# Autodesk Inventor assembly: Tarot 810 Reverse
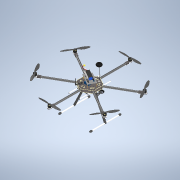
[picture p0: Inventor's stored thumbnail of the model, 180x180]
Saved by Autodesk Inventor 2020 (Build 240168000, 168)
## iProperties
Created: 2020-04-17
Part Number: Tarot 810 Reverse
Document SubType Name: Assembly
Designer: Muhyidin
Author: Muhyidin
## Documents named in this file (20)
- D:\ITS\BAYUCARAKA\PROYEK '19 - '20\Tarot 810\Tarot 810 Reverse.iam
- D:\ITS\BAYUCARAKA\PROYEK '19 - '20\Tarot 810\FRAME ATAS.ipt
- D:\ITS\BAYUCARAKA\PROYEK '19 - '20\Tarot 810\Arem2.iam
- D:\ITS\BAYUCARAKA\PROYEK '19 - '20\Tarot 810\FRAME BAWAH.ipt
- D:\ITS\BAYUCARAKA\PROYEK '19 - '20\Tarot 810\retractable-landing-gear-octocopter-1.snapshot.9\retract assy.iam
- D:\ITS\BAYUCARAKA\PROYEK '19 - '20\Tarot 810\ganjalan landing gear.ipt
- D:\ITS\BAYUCARAKA\PROYEK '19 - '20\Tarot 810\T-Motor U5.ipt
- D:\ITS\BAYUCARAKA\PROYEK '19 - '20\Tarot 810\antena_arm.ipt
- D:\ITS\BAYUCARAKA\PROYEK '19 - '20\Tarot 810\antena_GPS.ipt
- D:\ITS\BAYUCARAKA\PROYEK '19 - '20\Tarot 810\mounting_gps.ipt
- D:\ITS\BAYUCARAKA\PROYEK '19 - '20\Tarot 810\propeler.ipt
- D:\ITS\BAYUCARAKA\PROYEK '19 - '20\Tarot 810\Pixhawk.iam
- D:\ITS\BAYUCARAKA\PROYEK '19 - '20\Tarot 810\Rasberry_box_assembly.iam
- D:\ITS\BAYUCARAKA\PROYEK '19 - '20\Tarot 810\Distans Erkek M3x50mm YP-550.ipt
- D:\ITS\BAYUCARAKA\PROYEK '19 - '20\Tarot 810\Tempat Batere.ipt
- D:\ITS\BAYUCARAKA\PROYEK '19 - '20\Tarot 810\m3.ipt
- D:\ITS\BAYUCARAKA\PROYEK '19 - '20\Tarot 810\Telemetry.iam
- D:\ITS\BAYUCARAKA\PROYEK '19 - '20\Tarot 810\BATERIA.ipt
- D:\ITS\BAYUCARAKA\PROYEK '19 - '20\Tarot 810\bolt_atas.ipt
- D:\ITS\BAYUCARAKA\PROYEK '19 - '20\Tarot 810\mur M3.ipt
## Components (87 placed, 19 different names)
1. FRAME ATAS:1 — Rotational:1, Rotational:2, Rotational:3, Rotational:4, Rotational:5, Rotational:6, Rotational:17, Rotational:26, Rotational:28, Rotational:29, Rotational:30, Rotational:31, Rotational:32, Rigid:1, Rigid:2, Rigid:3, Rigid:4, Rigid:5, Rigid:6, Rigid:7, Rigid:8, Rigid:9, Rigid:10, Rigid:11, Rigid:12, Rigid:13, Rigid:14, Rigid:15, Rigid:16, Rigid:17, Rigid:18, Rigid:19, Rigid:20, Rigid:21, Rigid:22, Rigid:23, Rigid:24, Rigid:25
2. Arem2:1 [sub-assembly] — Rotational:1, Rotational:7, Rotational:12
3. Arem2:2 [sub-assembly] — Rotational:2, Rotational:11
4. Arem2:3 [sub-assembly] — Rotational:3, Rotational:13
5. Arem2:4 [sub-assembly] — Rotational:4, Rotational:14
6. Arem2:5 [sub-assembly] — Rotational:5, Rotational:15
7. Arem2:6 [sub-assembly] — Rotational:6, Rotational:16
8. FRAME BAWAH:1 — Rotational:7, Rotational:8, Rotational:9, Rotational:39, Rotational:40, Rotational:41, Rotational:42, Rotational:43, Rotational:44, Rotational:45, Rotational:46, Rotational:47, Rotational:48, Rotational:49, Rotational:50, Rotational:51, Rotational:52, Rotational:53, Rotational:54, Rotational:55, Rotational:56, Rotational:57, Rotational:58, Rotational:59, Rotational:60, Rotational:61, Rotational:62
9. retract assy:1 [sub-assembly] — Rotational:10
10. ganjalan landing gear:1 — Rotational:8, Rotational:10
11. ganjalan landing gear:2 — Rotational:9
12. T-Motor U5:1 — Rotational:11, Rotational:24
13. T-Motor U5:2 — Rotational:13, Rotational:20
14. T-Motor U5:3 — Rotational:14, Rotational:21
15. T-Motor U5:4 — Rotational:15, Rotational:22
16. T-Motor U5:5 — Rotational:16, Rotational:23
17. T-Motor U5:6 — Rotational:12, Rotational:25
18. antena_arm:1 — Rotational:18, Rotational:19
19. antena_GPS:1 — Rotational:19
20. mounting_gps:1 — Rotational:17, Rotational:18
21. propeler:1 — Rotational:20
22. propeler:2 — Rotational:21
23. propeler:3 — Rotational:22
24. propeler:4 — Rotational:23
25. propeler:5 — Rotational:24
26. propeler:6 — Rotational:25
27. Pixhawk:1 [sub-assembly] — Rotational:27
28. Rasberry_box_assembly:1 [sub-assembly] — Rotational:26, Rotational:27
29. Distans Erkek M3x50mm YP-550:1 — Rotational:28
30. Distans Erkek M3x50mm YP-550:2 — Rotational:29
31. Distans Erkek M3x50mm YP-550:3 — Rotational:31
32. Distans Erkek M3x50mm YP-550:4 — Rotational:30
33. Tempat Batere:1 — Rotational:32, Rotational:33, Rotational:34, Rotational:35, Rotational:36, Rotational:63
34. m3:1 — Rotational:35
35. m3:2 — Rotational:36
36. m3:3 — Rotational:34
37. m3:4 — Rotational:33
38. bolt_atas:1 — Rigid:12
39. bolt_atas:2 — Rigid:11
40. bolt_atas:3 — Rigid:9
41. bolt_atas:4 — Rigid:10
42. bolt_atas:5 — Rigid:8
43. bolt_atas:6 — Rigid:7
44. bolt_atas:7 — Rigid:6
45. bolt_atas:8 — Rigid:4
46. bolt_atas:9 — Rigid:5
47. bolt_atas:10 — Rigid:1
48. bolt_atas:11 — Rigid:3
49. bolt_atas:12 — Rigid:2
50. bolt_atas:13 — Rigid:13
51. bolt_atas:14 — Rigid:14
52. bolt_atas:15 — Rigid:15
53. bolt_atas:16 — Rigid:16
54. bolt_atas:17 — Rigid:17
55. bolt_atas:18 — Rigid:18
56. bolt_atas:19 — Rigid:19
57. bolt_atas:20 — Rigid:20
58. bolt_atas:21 — Rigid:21
59. bolt_atas:22 — Rigid:22
60. bolt_atas:23 — Rigid:23
61. bolt_atas:24 — Rigid:24
62. Telemetry:1 [sub-assembly] — Rigid:25
63. mur M3:1 — Rotational:41
64. mur M3:2 — Rotational:45
65. mur M3:3 — Rotational:50
66. mur M3:4 — Rotational:51
67. mur M3:5 — Rotational:46
68. mur M3:6 — Rotational:44
69. mur M3:7 — Rotational:57
70. mur M3:8 — Rotational:62
71. mur M3:9 — Rotational:59
72. mur M3:10 — Rotational:61
73. mur M3:11 — Rotational:47
74. mur M3:12 — Rotational:39
75. mur M3:13 — Rotational:40
76. mur M3:14 — Rotational:49
77. mur M3:16 — Rotational:58
78. mur M3:17 — Rotational:56
79. mur M3:18 — Rotational:53
80. mur M3:19 — Rotational:55
81. mur M3:21 — Rotational:60
82. mur M3:22 — Rotational:42
83. mur M3:23 — Rotational:43
84. mur M3:24 — Rotational:48
85. mur M3:25 — Rotational:54
86. mur M3:26 — Rotational:52
87. BATERIA:1 — Rotational:63
## Relationships (86: RevoluteJoint 61, WeldJoint 25)
- Rotational:1 [RevoluteJoint]: FRAME ATAS:1 ↔ Arem2:1
- Rotational:2 [RevoluteJoint]: FRAME ATAS:1 ↔ Arem2:2
- Rotational:3 [RevoluteJoint]: FRAME ATAS:1 ↔ Arem2:3
- Rotational:4 [RevoluteJoint]: FRAME ATAS:1 ↔ Arem2:4
- Rotational:5 [RevoluteJoint]: FRAME ATAS:1 ↔ Arem2:5
- Rotational:6 [RevoluteJoint]: FRAME ATAS:1 ↔ Arem2:6
- Rotational:7 [RevoluteJoint]: Arem2:1 ↔ FRAME BAWAH:1
- Rotational:8 [RevoluteJoint]: FRAME BAWAH:1 ↔ ganjalan landing gear:1
- Rotational:9 [RevoluteJoint]: FRAME BAWAH:1 ↔ ganjalan landing gear:2
- Rotational:10 [RevoluteJoint]: retract assy:1 ↔ ganjalan landing gear:1
- Rotational:11 [RevoluteJoint]: Arem2:2 ↔ T-Motor U5:1
- Rotational:12 [RevoluteJoint]: Arem2:1 ↔ T-Motor U5:6
- Rotational:13 [RevoluteJoint]: Arem2:3 ↔ T-Motor U5:2
- Rotational:14 [RevoluteJoint]: Arem2:4 ↔ T-Motor U5:3
- Rotational:15 [RevoluteJoint]: Arem2:5 ↔ T-Motor U5:4
- Rotational:16 [RevoluteJoint]: Arem2:6 ↔ T-Motor U5:5
- Rotational:17 [RevoluteJoint]: FRAME ATAS:1 ↔ mounting_gps:1
- Rotational:18 [RevoluteJoint]: antena_arm:1 ↔ mounting_gps:1
- Rotational:19 [RevoluteJoint] (-15 mm): antena_arm:1 ↔ antena_GPS:1
- Rotational:20 [RevoluteJoint]: T-Motor U5:2 ↔ propeler:1
- Rotational:21 [RevoluteJoint]: T-Motor U5:3 ↔ propeler:2
- Rotational:22 [RevoluteJoint]: T-Motor U5:4 ↔ propeler:3
- Rotational:23 [RevoluteJoint]: T-Motor U5:5 ↔ propeler:4
- Rotational:24 [RevoluteJoint]: T-Motor U5:1 ↔ propeler:5
- Rotational:25 [RevoluteJoint]: T-Motor U5:6 ↔ propeler:6
- Rotational:26 [RevoluteJoint]: FRAME ATAS:1 ↔ Rasberry_box_assembly:1
- Rotational:27 [RevoluteJoint]: Pixhawk:1 ↔ Rasberry_box_assembly:1
- Rotational:28 [RevoluteJoint]: FRAME ATAS:1 ↔ Distans Erkek M3x50mm YP-550:1
- Rotational:29 [RevoluteJoint]: FRAME ATAS:1 ↔ Distans Erkek M3x50mm YP-550:2
- Rotational:30 [RevoluteJoint]: FRAME ATAS:1 ↔ Distans Erkek M3x50mm YP-550:4
- Rotational:31 [RevoluteJoint]: FRAME ATAS:1 ↔ Distans Erkek M3x50mm YP-550:3
- Rotational:32 [RevoluteJoint] (50 mm): FRAME ATAS:1 ↔ Tempat Batere:1
- Rotational:33 [RevoluteJoint]: Tempat Batere:1 ↔ m3:4
- Rotational:34 [RevoluteJoint]: Tempat Batere:1 ↔ m3:3
- Rotational:35 [RevoluteJoint]: Tempat Batere:1 ↔ m3:1
- Rotational:36 [RevoluteJoint]: Tempat Batere:1 ↔ m3:2
- Rigid:1 [WeldJoint] (2 mm): FRAME ATAS:1 ↔ bolt_atas:10
- Rigid:2 [WeldJoint] (2 mm): FRAME ATAS:1 ↔ bolt_atas:12
- Rigid:3 [WeldJoint] (-2 mm): FRAME ATAS:1 ↔ bolt_atas:11
- Rigid:4 [WeldJoint] (-2 mm): FRAME ATAS:1 ↔ bolt_atas:8
- Rigid:5 [WeldJoint] (2 mm): FRAME ATAS:1 ↔ bolt_atas:9
- Rigid:6 [WeldJoint] (-2 mm): FRAME ATAS:1 ↔ bolt_atas:7
- Rigid:7 [WeldJoint] (-2 mm): FRAME ATAS:1 ↔ bolt_atas:6
- Rigid:8 [WeldJoint] (-2 mm): FRAME ATAS:1 ↔ bolt_atas:5
- Rigid:9 [WeldJoint] (-2 mm): FRAME ATAS:1 ↔ bolt_atas:3
- Rigid:10 [WeldJoint] (-2 mm): FRAME ATAS:1 ↔ bolt_atas:4
- Rigid:11 [WeldJoint] (2 mm): FRAME ATAS:1 ↔ bolt_atas:2
- Rigid:12 [WeldJoint] (2 mm): FRAME ATAS:1 ↔ bolt_atas:1
- Rigid:13 [WeldJoint] (-2 mm): FRAME ATAS:1 ↔ bolt_atas:13
- Rigid:14 [WeldJoint] (-2 mm): FRAME ATAS:1 ↔ bolt_atas:14
- Rigid:15 [WeldJoint] (-2 mm): FRAME ATAS:1 ↔ bolt_atas:15
- Rigid:16 [WeldJoint] (-2 mm): FRAME ATAS:1 ↔ bolt_atas:16
- Rigid:17 [WeldJoint] (2 mm): FRAME ATAS:1 ↔ bolt_atas:17
- Rigid:18 [WeldJoint] (-2 mm): FRAME ATAS:1 ↔ bolt_atas:18
- Rigid:19 [WeldJoint] (2 mm): FRAME ATAS:1 ↔ bolt_atas:19
- Rigid:20 [WeldJoint] (-2 mm): FRAME ATAS:1 ↔ bolt_atas:20
- Rigid:21 [WeldJoint] (2 mm): FRAME ATAS:1 ↔ bolt_atas:21
- Rigid:22 [WeldJoint] (-2 mm): FRAME ATAS:1 ↔ bolt_atas:22
- Rigid:23 [WeldJoint] (-2 mm): FRAME ATAS:1 ↔ bolt_atas:23
- Rigid:24 [WeldJoint] (-2 mm): FRAME ATAS:1 ↔ bolt_atas:24
- Rigid:25 [WeldJoint]: FRAME ATAS:1 ↔ Telemetry:1
- Rotational:39 [RevoluteJoint]: FRAME BAWAH:1 ↔ mur M3:12
- Rotational:40 [RevoluteJoint]: FRAME BAWAH:1 ↔ mur M3:13
- Rotational:41 [RevoluteJoint]: FRAME BAWAH:1 ↔ mur M3:1
- Rotational:42 [RevoluteJoint]: FRAME BAWAH:1 ↔ mur M3:22
- Rotational:43 [RevoluteJoint]: FRAME BAWAH:1 ↔ mur M3:23
- Rotational:44 [RevoluteJoint]: FRAME BAWAH:1 ↔ mur M3:6
- Rotational:45 [RevoluteJoint]: FRAME BAWAH:1 ↔ mur M3:2
- Rotational:46 [RevoluteJoint]: FRAME BAWAH:1 ↔ mur M3:5
- Rotational:47 [RevoluteJoint]: FRAME BAWAH:1 ↔ mur M3:11
- Rotational:48 [RevoluteJoint]: FRAME BAWAH:1 ↔ mur M3:24
- Rotational:49 [RevoluteJoint]: FRAME BAWAH:1 ↔ mur M3:14
- Rotational:50 [RevoluteJoint]: FRAME BAWAH:1 ↔ mur M3:3
- Rotational:51 [RevoluteJoint]: FRAME BAWAH:1 ↔ mur M3:4
- Rotational:52 [RevoluteJoint]: FRAME BAWAH:1 ↔ mur M3:26
- Rotational:53 [RevoluteJoint]: FRAME BAWAH:1 ↔ mur M3:18
- Rotational:54 [RevoluteJoint]: FRAME BAWAH:1 ↔ mur M3:25
- Rotational:55 [RevoluteJoint]: FRAME BAWAH:1 ↔ mur M3:19
- Rotational:56 [RevoluteJoint]: FRAME BAWAH:1 ↔ mur M3:17
- Rotational:57 [RevoluteJoint]: FRAME BAWAH:1 ↔ mur M3:7
- Rotational:58 [RevoluteJoint]: FRAME BAWAH:1 ↔ mur M3:16
- Rotational:59 [RevoluteJoint]: FRAME BAWAH:1 ↔ mur M3:9
- Rotational:60 [RevoluteJoint]: FRAME BAWAH:1 ↔ mur M3:21
- Rotational:61 [RevoluteJoint]: FRAME BAWAH:1 ↔ mur M3:10
- Rotational:62 [RevoluteJoint]: FRAME BAWAH:1 ↔ mur M3:8
- Rotational:63 [RevoluteJoint]: Tempat Batere:1 ↔ BATERIA:1
